# Autodesk Inventor assembly: Motor Mount with Motor
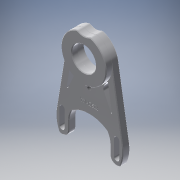
[picture p0: Inventor's stored thumbnail of the model, 180x180]
Saved by Autodesk Inventor 2019.3 (Build 233278000, 278)
## iProperties
Created: 2019-03-01
Part Number: Motor Mount with Motor
Document SubType Name: Assembly
Designer: Petar
Mass: 37.7633 g
Surface Area: 102.459 cm^2
Volume: 12.7696 cm^3
Density: 2.95729 g/cm^3
Author: Petar
## Documents named in this file (3)
- D:\OMG\E-Board\CAD\Inventor\Motor Mount - 225 - ABS.iam
- D:\OMG\E-Board\CAD\Inventor\Mechanical Components\Motor Holder v3 - 225 - ABS.ipt
- D:\OMG\E-Board\CAD\Inventor\Mechanical Components\Motor Mount - ABS.ipt
## Components (2 placed, 2 different names)
1. Motor Holder v3 - 225 - ABS:1 — Mate:2, Rigid:1
2. Motor Mount - ABS:1 — Mate:2, Rigid:1
## Relationships (2: Mate 1, WeldJoint 1)
- Mate:2: Motor Holder v3 - 225 - ABS:1 ↔ Motor Mount - ABS:1
- Rigid:1 [WeldJoint]: Motor Holder v3 - 225 - ABS:1 ↔ Motor Mount - ABS:1
